# Autodesk Inventor assembly: KneeUnit
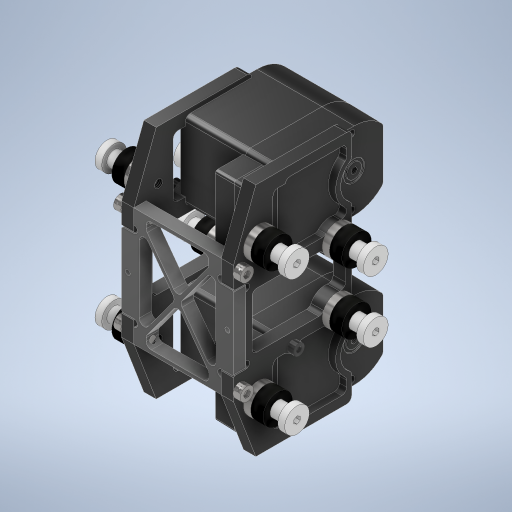
[picture p0: Inventor's stored thumbnail of the model, 512x512]
Saved by Autodesk Inventor 2024.2 (Build 282272000, 272)
## iProperties
Created: 2024-01-06
Part Number: KneeUnit
Document SubType Name: Assembly
Designer: Masato Kubotera
Mass: 357.633 g
Surface Area: 532.224 cm^2
Volume: 146.435 cm^3
Author: Masato Kubotera
## Documents named in this file (11)
- C:\Users\masato\OneDrive - Chiba Institute of Technology\CIT Brains\RoboCup2024\Mechanic\SUSTAINA-OP2\NativeFiles\Boby\LowerLimb\Legs\Knees\KneeUnit.iam
- C:\Users\masato\OneDrive - Chiba Institute of Technology\CIT Brains\RoboCup2024\Mechanic\SUSTAINA-OP2\NativeFiles\Boby\LowerLimb\Legs\Knees\KneeHornSideFrame.ipt
- C:\Users\masato\OneDrive - Chiba Institute of Technology\CIT Brains\RoboCup2024\Mechanic\SUSTAINA-OP2\NativeFiles\Boby\LowerLimb\Legs\Knees\KneeIdlerSideFrame.ipt
- C:\Users\masato\OneDrive - Chiba Institute of Technology\CIT Brains\RoboCup2024\Mechanic\SUSTAINA-OP2\NativeFiles\Boby\COTS\Actuators\PMX-SCR-9203HV.ipt
- C:\Users\masato\OneDrive - Chiba Institute of Technology\CIT Brains\RoboCup2024\Mechanic\SUSTAINA-OP2\NativeFiles\Boby\COTS\Washers\Metal\UUW-0412-30H.ipt
- C:\Users\masato\OneDrive - Chiba Institute of Technology\CIT Brains\RoboCup2024\Mechanic\SUSTAINA-OP2\NativeFiles\Boby\COTS\Washers\Resin\CC-0612-50B.ipt
- C:\Users\masato\OneDrive - Chiba Institute of Technology\CIT Brains\RoboCup2024\Mechanic\SUSTAINA-OP2\NativeFiles\Boby\COTS\Screws\CapScrew\FC-2615EB.ipt
- C:\Users\masato\OneDrive - Chiba Institute of Technology\CIT Brains\RoboCup2024\Mechanic\SUSTAINA-OP2\NativeFiles\Boby\COTS\Screws\CapScrew\FC-2620EB.ipt
- C:\Users\masato\OneDrive - Chiba Institute of Technology\CIT Brains\RoboCup2024\Mechanic\SUSTAINA-OP2\NativeFiles\Boby\LowerLimb\Legs\Knees\KneeBraceFrame.ipt
- C:\Users\masato\OneDrive - Chiba Institute of Technology\CIT Brains\RoboCup2024\Mechanic\SUSTAINA-OP2\NativeFiles\Boby\COTS\Screws\CapScrew\UC-0310.ipt
- C:\Users\masato\OneDrive - Chiba Institute of Technology\CIT Brains\RoboCup2024\Mechanic\SUSTAINA-OP2\NativeFiles\Boby\COTS\Screws\ScrewsWithShoulder\DBSY4-10-6.ipt
## Components (37 placed, 10 different names)
1. KneeHornSideFrame:1 — Mate:1, Angle:1, Insert:2, Insert:3, Insert:9, Insert:18, Insert:19, Insert:20, Insert:26, Insert:27, Insert:51, Insert:52, Insert:55, Insert:56
2. KneeIdlerSideFrame:1 — Insert:6, Insert:7, Insert:21, Insert:22, Insert:23, Insert:24, Insert:30, Insert:31, Insert:49, Insert:50, Insert:53, Insert:54
3. KneeBraceFrame:1 — Insert:49, Insert:50, Insert:51, Insert:52, Flush:1
4. PMX-SCR-9203HV:1 — Insert:2, Insert:6, Angle:2
5. PMX-SCR-9203HV:2 — Insert:3, Insert:7, Angle:3
6. UC-0310:1 — Insert:53
7. UC-0310:2 — Insert:54
8. UC-0310:3 — Insert:55
9. UC-0310:4 — Insert:56
10. FC-2620EB:2 — Insert:30
11. FC-2620EB:3 — Insert:31
12. FC-2615EB:2 — Insert:26
13. FC-2615EB:3 — Insert:27
14. CC-0612-50B:1 — Insert:10
15. CC-0612-50B:2
16. CC-0612-50B:3
17. CC-0612-50B:4
18. CC-0612-50B:6
19. CC-0612-50B:5
20. CC-0612-50B:7
21. CC-0612-50B:8
22. UUW-0412-30H:1 — Insert:9, Insert:10, Insert:41
23. UUW-0412-30H:2 — Insert:18, Insert:42
24. UUW-0412-30H:3 — Insert:19, Insert:43
25. UUW-0412-30H:4 — Insert:20, Insert:44
26. UUW-0412-30H:5 — Insert:21, Insert:45
27. UUW-0412-30H:6 — Insert:22, Insert:46
28. UUW-0412-30H:7 — Insert:23, Insert:47
29. UUW-0412-30H:8 — Insert:24, Insert:48
30. DBSY4-10-6:1 — Insert:41
31. DBSY4-10-6:2 — Insert:42
32. DBSY4-10-6:3 — Insert:43
33. DBSY4-10-6:4 — Insert:44
34. DBSY4-10-6:5 — Insert:45
35. DBSY4-10-6:6 — Insert:46
36. DBSY4-10-6:7 — Insert:47
37. DBSY4-10-6:8 — Insert:48
## Relationships (45: Insert 40, Angle 3, Mate 1, Flush 1)
- Mate:1: KneeHornSideFrame:1
- Angle:1 (0 deg): KneeHornSideFrame:1
- Flush:1: KneeBraceFrame:1
- Insert:2: KneeHornSideFrame:1 ↔ PMX-SCR-9203HV:1
- Insert:3: KneeHornSideFrame:1 ↔ PMX-SCR-9203HV:2
- Insert:6: KneeIdlerSideFrame:1 ↔ PMX-SCR-9203HV:1
- Insert:7: KneeIdlerSideFrame:1 ↔ PMX-SCR-9203HV:2
- Insert:9: KneeHornSideFrame:1 ↔ UUW-0412-30H:1
- Insert:10: CC-0612-50B:1 ↔ UUW-0412-30H:1
- [Insert]: CC-0612-50B:2 ↔ UUW-0412-30H:2
- [Insert]: CC-0612-50B:3 ↔ UUW-0412-30H:3
- [Insert]: CC-0612-50B:4 ↔ UUW-0412-30H:4
- [Insert]: CC-0612-50B:5 ↔ UUW-0412-30H:5
- [Insert]: CC-0612-50B:6 ↔ UUW-0412-30H:6
- [Insert]: CC-0612-50B:7 ↔ UUW-0412-30H:7
- [Insert]: CC-0612-50B:8 ↔ UUW-0412-30H:8
- Insert:18: KneeHornSideFrame:1 ↔ UUW-0412-30H:2
- Insert:19: KneeHornSideFrame:1 ↔ UUW-0412-30H:3
- Insert:20: KneeHornSideFrame:1 ↔ UUW-0412-30H:4
- Insert:21: KneeIdlerSideFrame:1 ↔ UUW-0412-30H:5
- Insert:22: KneeIdlerSideFrame:1 ↔ UUW-0412-30H:6
- Insert:23: KneeIdlerSideFrame:1 ↔ UUW-0412-30H:7
- Insert:24: KneeIdlerSideFrame:1 ↔ UUW-0412-30H:8
- Insert:26: KneeHornSideFrame:1 ↔ FC-2615EB:2
- Insert:27: KneeHornSideFrame:1 ↔ FC-2615EB:3
- Insert:30: KneeIdlerSideFrame:1 ↔ FC-2620EB:2
- Insert:31: KneeIdlerSideFrame:1 ↔ FC-2620EB:3
- Insert:41: UUW-0412-30H:1 ↔ DBSY4-10-6:1
- Insert:42: UUW-0412-30H:2 ↔ DBSY4-10-6:2
- Insert:43: UUW-0412-30H:3 ↔ DBSY4-10-6:3
- Insert:44: UUW-0412-30H:4 ↔ DBSY4-10-6:4
- Insert:45: UUW-0412-30H:5 ↔ DBSY4-10-6:5
- Insert:46: UUW-0412-30H:6 ↔ DBSY4-10-6:6
- Insert:47: UUW-0412-30H:7 ↔ DBSY4-10-6:7
- Insert:48: UUW-0412-30H:8 ↔ DBSY4-10-6:8
- Insert:49: KneeIdlerSideFrame:1 ↔ KneeBraceFrame:1
- Insert:50: KneeIdlerSideFrame:1 ↔ KneeBraceFrame:1
- Insert:51: KneeHornSideFrame:1 ↔ KneeBraceFrame:1
- Insert:52: KneeHornSideFrame:1 ↔ KneeBraceFrame:1
- Insert:53: KneeIdlerSideFrame:1 ↔ UC-0310:1
- Insert:54: KneeIdlerSideFrame:1 ↔ UC-0310:2
- Insert:55: KneeHornSideFrame:1 ↔ UC-0310:3
- Insert:56: KneeHornSideFrame:1 ↔ UC-0310:4
- Angle:2 (0 deg): PMX-SCR-9203HV:1
- Angle:3 (0 deg): PMX-SCR-9203HV:2
## Named parameters: d13_d12 = 0 mm, d14_d12 = 0 mm, d15_d12 = 0 mm, d16_d12 = 0 mm, d17_d12 = 0 mm, d18_d12 = 0 mm, d19_d12 = 0 mm
